# Autodesk Inventor assembly: Assembly_Cube_M12_VCAmount_Kinematic_Mirror_90
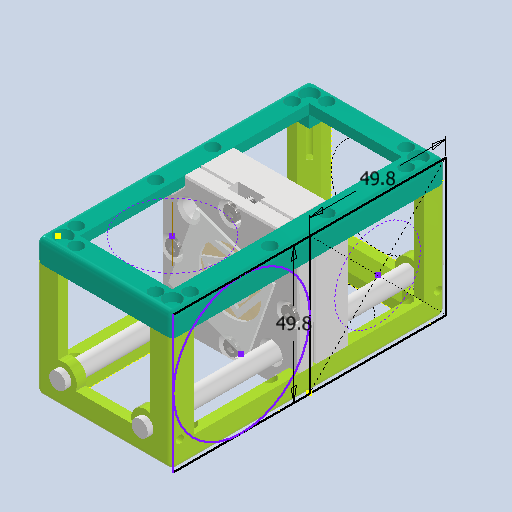
[picture p0: Inventor's stored thumbnail of the model, 512x512]
Saved by Autodesk Inventor 2022.3 (Build 263350000, 350)
## iProperties
Created: 2022-06-27
Part Number: Assembly_Cube_M12_VCAmount_Kinematic_Mirror_90
Document SubType Name: Assembly
Designer: bingoeleda
Author: bingoeleda
## Documents named in this file (6)
- G:\My Drive\ASP - M.Sc. Photonics\Practical Modules\MODULE 4 - Master Thesis\2.Experiments\Modules\11.Reference_Mirror_Module\Reference_Mirror_with_UC2-VCA_Module\Assembly_Cube_VCA_mirror.iam
- G:\My Drive\ASP - M.Sc. Photonics\Practical Modules\MODULE 4 - Master Thesis\2.Experiments\Modules\2.Base_Cube\Base_Cube_3DP\Base_Cube_3DP_2x1\with RODS\10_Cube_2x1_v3.ipt
- G:\My Drive\ASP - M.Sc. Photonics\Practical Modules\MODULE 4 - Master Thesis\2.Experiments\Modules\2.Base_Cube\Base_Cube_3DP\Base_Cube_3DP_2x1\with RODS\10_Lid_2x1_v3.ipt
- G:\My Drive\ASP - M.Sc. Photonics\Practical Modules\MODULE 4 - Master Thesis\2.Experiments\Modules\11.Reference_Mirror_Module\Reference_Mirror_with_UC2-VCA_Module\00_Thorlabs_Rod_6mm.ipt
- G:\My Drive\ASP - M.Sc. Photonics\Practical Modules\MODULE 4 - Master Thesis\2.Experiments\Modules\11.Reference_Mirror_Module\Reference_Mirror_with_UC2-VCA_Module\Assembly_Cube_VCA_v0.iam
- C:\Users\bingoeleda\Documents\Inventor\Content Center Files\R2022\en-US\DIN 912\DIN 912 - M3 x 0.5 x 6 x 4.75.ipt
## Components (9 placed, 5 different names)
1. 10_Cube_2x1_v3:1 — Rotational:1, Rigid:1, Rigid:2, Rotational:2, Rotational:3, Rotational:4, Rotational:5
2. 10_Lid_2x1_v3:1 — Rotational:1
3. 00_Thorlabs_Rod_6mm:1 — Rigid:2, Rigid:3
4. 00_Thorlabs_Rod_6mm:2 — Rigid:1
5. Assembly_Cube_VCA_v0:1 [sub-assembly] — Rigid:3
6. DIN 912 - replaced by DIN EN ISO 4762 M3 x 6:1 — Rotational:5
7. DIN 912 - replaced by DIN EN ISO 4762 M3 x 6:2 — Rotational:4
8. DIN 912 - replaced by DIN EN ISO 4762 M3 x 6:3 — Rotational:2
9. DIN 912 - replaced by DIN EN ISO 4762 M3 x 6:4 — Rotational:3
## Relationships (8: RevoluteJoint 5, WeldJoint 3)
- Rotational:1 [RevoluteJoint]: 10_Cube_2x1_v3:1 ↔ 10_Lid_2x1_v3:1
- Rigid:1 [WeldJoint] (-2 mm): 10_Cube_2x1_v3:1 ↔ 00_Thorlabs_Rod_6mm:2
- Rigid:2 [WeldJoint] (-2 mm): 10_Cube_2x1_v3:1 ↔ 00_Thorlabs_Rod_6mm:1
- Rigid:3 [WeldJoint]: 00_Thorlabs_Rod_6mm:1 ↔ Assembly_Cube_VCA_v0:1
- Rotational:2 [RevoluteJoint]: 10_Cube_2x1_v3:1 ↔ DIN 912 - replaced by DIN EN ISO 4762 M3 x 6:3
- Rotational:3 [RevoluteJoint]: 10_Cube_2x1_v3:1 ↔ DIN 912 - replaced by DIN EN ISO 4762 M3 x 6:4
- Rotational:4 [RevoluteJoint]: 10_Cube_2x1_v3:1 ↔ DIN 912 - replaced by DIN EN ISO 4762 M3 x 6:2
- Rotational:5 [RevoluteJoint]: 10_Cube_2x1_v3:1 ↔ DIN 912 - replaced by DIN EN ISO 4762 M3 x 6:1
